# Autodesk Inventor assembly: Wrist 2
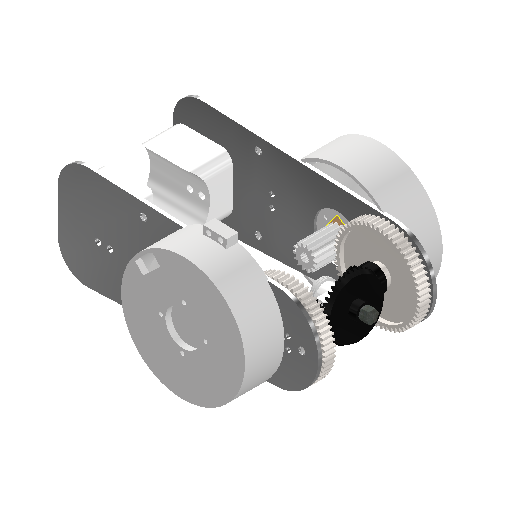
[picture p0: Inventor's stored thumbnail of the model, 512x512]
Saved by Autodesk Inventor 2025.1 (Build 291241020, 241B)
## iProperties
Created: 2022-09-21
Part Number: Wrist 2
Document SubType Name: Assembly
Designer: caden
Mass: 1673.41 g
Surface Area: 3755.26 cm^2
Volume: 1174.27 cm^3
Density: 1.42507 g/cm^3
Author: caden
## Documents named in this file (17)
- C:\Users\t205b\OneDrive\Documents\Github\BehrendURCMechanical\CAD\Apparatus\ARM MAIN\WRIST\Wrist 2.iam
- C:\Users\t205b\OneDrive\Documents\Github\BehrendURCMechanical\CAD\Apparatus\ARM MAIN\WRIST\Wrist Side Brase.ipt
- C:\Users\t205b\OneDrive\Documents\Github\BehrendURCMechanical\CAD\Apparatus\ARM MAIN\WRIST\Pipe Holder.ipt
- C:\Users\t205b\OneDrive\Documents\Github\BehrendURCMechanical\CAD\Apparatus\ARM MAIN\WRIST\Space.ipt
- C:\Users\t205b\OneDrive\Documents\Github\BehrendURCMechanical\CAD\Apparatus\ARM MAIN\WRIST\Gears\am-2620 40t 1-25mod bevel gear.ipt
- C:\Users\t205b\OneDrive\Documents\Github\BehrendURCMechanical\CAD\Apparatus\ARM MAIN\WRIST\Gears\Gear assembly.iam
- C:\Users\t205b\OneDrive\Documents\Github\BehrendURCMechanical\CAD\Apparatus\ARM MAIN\Hardware\57155K621_Flanged Ball Bearing.ipt
- C:\Users\t205b\OneDrive\Documents\Github\BehrendURCMechanical\CAD\Apparatus\ARM MAIN\WRIST\Gears\Gear Shaft connector.ipt
- C:\Users\t205b\OneDrive\Documents\Github\BehrendURCMechanical\CAD\Apparatus\ARM MAIN\Hardware\7804K116_Stainless Steel Ball Bearing.ipt
- C:\Users\t205b\OneDrive\Documents\Github\BehrendURCMechanical\CAD\Apparatus\ARM MAIN\WRIST\Gears\bevel gear shaft connector for versaball.ipt
- C:\Users\t205b\OneDrive\Documents\Github\BehrendURCMechanical\CAD\Apparatus\ARM MAIN\Hardware\6389K723_Light Duty Dry-Running Nylon Sleeve Bearing.ipt
- C:\Users\t205b\OneDrive\Documents\Github\BehrendURCMechanical\CAD\Apparatus\ARM MAIN\Hardware\5909K3_Needle-Roller Thrust Bearing.ipt
- C:\Users\t205b\OneDrive\Documents\Github\BehrendURCMechanical\CAD\Apparatus\ARM MAIN\WRIST\EAGLE POWER 8308.ipt
- C:\Users\t205b\OneDrive\Documents\Github\BehrendURCMechanical\CAD\Apparatus\ARM MAIN\Hardware\5909K295_1 mm Thick Washer for 8 mm Shaft Diameter Needle-Roller Thrust Bearing.ipt
- C:\Users\t205b\OneDrive\Documents\Github\BehrendURCMechanical\CAD\Apparatus\ARM MAIN\Hardware\99178A104_Heavy Duty Side-Mount External Retaining Ring.ipt
- C:\Users\t205b\OneDrive\Documents\Github\BehrendURCMechanical\CAD\Apparatus\ARM MAIN\WRIST\MotorAdapter.ipt
- C:\Users\t205b\OneDrive\Documents\Github\BehrendURCMechanical\CAD\Apparatus\ARM MAIN\WRIST\MotorHouse.ipt
## Components (29 placed, 16 different names)
1. Wrist Side Brase:1 — Mate:1, Mate:2, Mate:3, Mate:6, Mate:7, Mate:45, Mate:46, Mate:47, Mate:59, Mate:60, Mate:61, Cylindrical:1, Cylindrical:3
2. Wrist Side Brase:2 — Rotational:2, Insert:1, Cylindrical:1, Cylindrical:2, Rotational:3
3. Pipe Holder:1 — Insert:1, Cylindrical:2, Cylindrical:3
4. Pipe Holder:2 — Mate:45, Mate:46, Mate:47
5. Space:1 — Mate:27, Mate:32, Flush:5, Mate:48, Mate:49, Flush:7, Mate:51, Mate:62, Mate:63, Mate:64
6. Gear assembly:1 [sub-assembly] — Mate:17, Mate:18, Mate:19
7. Gear assembly:2 [sub-assembly] — Mate:14, Mate:20, Mate:21, Rotational:3, Rotational:4
8. am-2620 40t 1-25mod bevel gear:1 — Mate:48
9. 57155K621_Flanged Ball Bearing:1 — Mate:6, Mate:7, Mate:12, Mate:13, Mate:19
10. 57155K621_Flanged Ball Bearing:2 — Mate:10, Mate:11, Mate:21
11. Gear Shaft connector:1 — Mate:10, Mate:11, Mate:14, Mate:20, Mate:67
12. Gear Shaft connector:2 — Mate:12, Mate:13, Mate:17, Mate:18, Mate:66
13. am-2620 40t 1-25mod bevel gear:2 — Mate:49
14. 7804K116_Stainless Steel Ball Bearing:2 — Mate:32, Flush:5
15. 6389K723_Light Duty Dry-Running Nylon Sleeve Bearing:1 — Flush:7, Rotational:4
16. 6389K723_Light Duty Dry-Running Nylon Sleeve Bearing:2
17. bevel gear shaft connector for versaball:1 — Mate:68, Mate:69
18. 5909K295_1 mm Thick Washer for 8 mm Shaft Diameter Needle-Roller Thrust Bearing:2 — Mate:62, Mate:63, Tangent:1
19. 5909K3_Needle-Roller Thrust Bearing:1 — Mate:51, Tangent:1, Tangent:2
20. 99178A104_Heavy Duty Side-Mount External Retaining Ring:1 — Mate:68, Mate:69, Mate:70
21. 99178A104_Heavy Duty Side-Mount External Retaining Ring:2 — Mate:67
22. 99178A104_Heavy Duty Side-Mount External Retaining Ring:3 — Mate:66
23. EAGLE POWER 8308:1 — Rotational:1, Rotational:2, Rotational:7
24. EAGLE POWER 8308:2 — Mate:59, Mate:60, Mate:61, Rotational:5, Rotational:6
25. 5909K295_1 mm Thick Washer for 8 mm Shaft Diameter Needle-Roller Thrust Bearing:1 — Tangent:2, Mate:64, Mate:70
26. MotorAdapter:1 — Rotational:1
27. MotorAdapter:2 — Rotational:5
28. MotorHouse:1 — Rotational:6
29. MotorHouse:2 — Rotational:7
## Relationships (59: Mate 43, RevoluteJoint 7, Flush 3, CylindricalJoint 3, Tangent 2, Insert 1)
- Mate:1: Wrist Side Brase:1
- Mate:2 (49.5 mm): Wrist Side Brase:1
- Mate:3: Wrist Side Brase:1
- Mate:6: Wrist Side Brase:1 ↔ 57155K621_Flanged Ball Bearing:1
- Mate:7: Wrist Side Brase:1 ↔ 57155K621_Flanged Ball Bearing:1
- Mate:10: 57155K621_Flanged Ball Bearing:2 ↔ Gear Shaft connector:1
- Mate:11: 57155K621_Flanged Ball Bearing:2 ↔ Gear Shaft connector:1
- Mate:12: 57155K621_Flanged Ball Bearing:1 ↔ Gear Shaft connector:2
- Mate:13: 57155K621_Flanged Ball Bearing:1 ↔ Gear Shaft connector:2
- Mate:14: Gear assembly:2 ↔ Gear Shaft connector:1
- Mate:17: Gear assembly:1 ↔ Gear Shaft connector:2
- Mate:18: Gear assembly:1 ↔ Gear Shaft connector:2
- Mate:19: Gear assembly:1 ↔ 57155K621_Flanged Ball Bearing:1
- Mate:20: Gear assembly:2 ↔ Gear Shaft connector:1
- Mate:21: Gear assembly:2 ↔ 57155K621_Flanged Ball Bearing:2
- Mate:27: Space:1
- [Mate]: 6389K723_Light Duty Dry-Running Nylon Sleeve Bearing:1 ↔ 6389K723_Light Duty Dry-Running Nylon Sleeve Bearing:2
- [Flush]: Space:1 ↔ 6389K723_Light Duty Dry-Running Nylon Sleeve Bearing:2
- [Mate]: Space:1 ↔ 6389K723_Light Duty Dry-Running Nylon Sleeve Bearing:2
- [Mate]: Gear Shaft connector:2 ↔ 6389K723_Light Duty Dry-Running Nylon Sleeve Bearing:2
- Mate:32: Space:1 ↔ 7804K116_Stainless Steel Ball Bearing:2
- Flush:5: Space:1 ↔ 7804K116_Stainless Steel Ball Bearing:2
- [Mate]: 7804K116_Stainless Steel Ball Bearing:2 ↔ bevel gear shaft connector for versaball:1
- [Mate]: Space:1 ↔ bevel gear shaft connector for versaball:1
- [Mate]: am-2620 40t 1-25mod bevel gear:1 ↔ bevel gear shaft connector for versaball:1
- [Mate]: am-2620 40t 1-25mod bevel gear:1 ↔ bevel gear shaft connector for versaball:1
- Mate:45: Wrist Side Brase:1 ↔ Pipe Holder:2
- Mate:46: Wrist Side Brase:1 ↔ Pipe Holder:2
- Mate:47: Wrist Side Brase:1 ↔ Pipe Holder:2
- Mate:48 (1.25 mm): Space:1 ↔ am-2620 40t 1-25mod bevel gear:1
- Mate:49 (1.25 mm): Space:1 ↔ am-2620 40t 1-25mod bevel gear:2
- Flush:7: Space:1 ↔ 6389K723_Light Duty Dry-Running Nylon Sleeve Bearing:1
- Mate:51: Space:1 ↔ 5909K3_Needle-Roller Thrust Bearing:1
- [Mate]: Gear Shaft connector:1 ↔ 99178A104_Heavy Duty Side-Mount External Retaining Ring:2
- [Mate]: Gear Shaft connector:2 ↔ 99178A104_Heavy Duty Side-Mount External Retaining Ring:3
- Mate:59: Wrist Side Brase:1 ↔ EAGLE POWER 8308:2
- Mate:60: Wrist Side Brase:1 ↔ EAGLE POWER 8308:2
- Mate:61: Wrist Side Brase:1 ↔ EAGLE POWER 8308:2
- Mate:62: Space:1 ↔ 5909K295_1 mm Thick Washer for 8 mm Shaft Diameter Needle-Roller Thrust Bearing:2
- Mate:63: Space:1 ↔ 5909K295_1 mm Thick Washer for 8 mm Shaft Diameter Needle-Roller Thrust Bearing:2
- Tangent:1: 5909K295_1 mm Thick Washer for 8 mm Shaft Diameter Needle-Roller Thrust Bearing:2 ↔ 5909K3_Needle-Roller Thrust Bearing:1
- Tangent:2: 5909K3_Needle-Roller Thrust Bearing:1 ↔ 5909K295_1 mm Thick Washer for 8 mm Shaft Diameter Needle-Roller Thrust Bearing:1
- Mate:64: Space:1 ↔ 5909K295_1 mm Thick Washer for 8 mm Shaft Diameter Needle-Roller Thrust Bearing:1
- Mate:66: Gear Shaft connector:2 ↔ 99178A104_Heavy Duty Side-Mount External Retaining Ring:3
- Mate:67: Gear Shaft connector:1 ↔ 99178A104_Heavy Duty Side-Mount External Retaining Ring:2
- Mate:68: bevel gear shaft connector for versaball:1 ↔ 99178A104_Heavy Duty Side-Mount External Retaining Ring:1
- Mate:69: bevel gear shaft connector for versaball:1 ↔ 99178A104_Heavy Duty Side-Mount External Retaining Ring:1
- Mate:70: 99178A104_Heavy Duty Side-Mount External Retaining Ring:1 ↔ 5909K295_1 mm Thick Washer for 8 mm Shaft Diameter Needle-Roller Thrust Bearing:1
- Rotational:1 [RevoluteJoint]: EAGLE POWER 8308:1 ↔ MotorAdapter:1
- Rotational:2 [RevoluteJoint]: Wrist Side Brase:2 ↔ EAGLE POWER 8308:1
- Insert:1: Wrist Side Brase:2 ↔ Pipe Holder:1
- Cylindrical:1: Wrist Side Brase:1 ↔ Wrist Side Brase:2
- Cylindrical:2: Wrist Side Brase:2 ↔ Pipe Holder:1
- Cylindrical:3: Wrist Side Brase:1 ↔ Pipe Holder:1
- Rotational:3 [RevoluteJoint]: Wrist Side Brase:2 ↔ Gear assembly:2
- Rotational:4 [RevoluteJoint]: Gear assembly:2 ↔ 6389K723_Light Duty Dry-Running Nylon Sleeve Bearing:1
- Rotational:5 [RevoluteJoint]: EAGLE POWER 8308:2 ↔ MotorAdapter:2
- Rotational:6 [RevoluteJoint]: EAGLE POWER 8308:2 ↔ MotorHouse:1
- Rotational:7 [RevoluteJoint]: EAGLE POWER 8308:1 ↔ MotorHouse:2
